# Autodesk Inventor assembly: LeftTorsoSideUnit
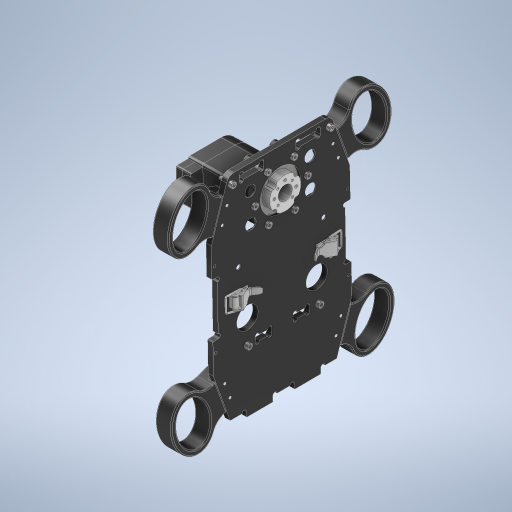
[picture p0: Inventor's stored thumbnail of the model, 512x512]
Saved by Autodesk Inventor 2024.2 (Build 282272000, 272)
## iProperties
Created: 2024-06-05
Part Number: LeftTorsoSideUnit
Document SubType Name: Assembly
Designer: Masato Kubotera
Author: Masato Kubotera
## Documents named in this file (3)
- D:\OneDrive - Chiba Institute of Technology\CIT Brains\RoboCup2024\Mechanic\SUSTAINA-OP2-DEV\NativeFiles\Boby\Torso\LeftTorsoSideUnit.iam
- D:\OneDrive - Chiba Institute of Technology\CIT Brains\RoboCup2024\Mechanic\SUSTAINA-OP2-DEV\NativeFiles\Boby\Torso\TorsoSideBaseUnit.iam
- D:\OneDrive - Chiba Institute of Technology\CIT Brains\RoboCup2024\Mechanic\SUSTAINA-OP2-DEV\NativeFiles\Boby\UpperLimb\Shoulders\LeftShoulderBearingUnit.iam
## Components (2 placed, 2 different names)
1. TorsoSideBaseUnit:1 [sub-assembly] — Flush:1, Flush:2, Flush:3, Insert:1, Insert:2
2. LeftShoulderBearingUnit:1 [sub-assembly] — Insert:1, Insert:2
## Relationships (5: Flush 3, Insert 2)
- Flush:1: TorsoSideBaseUnit:1
- Flush:2: TorsoSideBaseUnit:1
- Flush:3: TorsoSideBaseUnit:1
- Insert:1: TorsoSideBaseUnit:1 ↔ LeftShoulderBearingUnit:1
- Insert:2: TorsoSideBaseUnit:1 ↔ LeftShoulderBearingUnit:1
